# Autodesk Inventor assembly: GE-13027
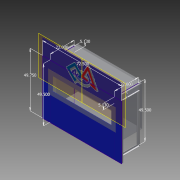
[picture p0: Inventor's stored thumbnail of the model, 180x180]
Saved by Autodesk Inventor 2013 (Build 170138000, 138)
## iProperties
Created: 2013-01-04
Part Number: GE-13027
Document SubType Name: Assembly
Designer: Phillip
Author: Phillip
## Documents named in this file (11)
- E:\Data Folder\FIRST 2013\FIRST KOP\FIRST Arena 2013\Feeder Goal Station\GE-13027.iam
- E:\Data Folder\FIRST 2013\FIRST KOP\FIRST Arena 2013\Feeder Goal Station\GE-13029.ipt
- E:\Data Folder\FIRST 2013\FIRST KOP\FIRST Arena 2013\Feeder Goal Station\GE-13013B.ipt
- E:\Data Folder\FIRST 2013\FIRST KOP\FIRST Arena 2013\Feeder Goal Station\GE-13013BLogo.ipt
- E:\Data Folder\FIRST 2013\FIRST KOP\FIRST Arena 2013\Feeder Goal Station\GE-13066.iam
- E:\Data Folder\FIRST 2013\FIRST KOP\FIRST Arena 2013\Feeder Goal Station\GE-13031.ipt
- E:\Data Folder\FIRST 2013\FIRST KOP\FIRST Arena 2013\Feeder Goal Station\box_middlegoal.ipt
- E:\Data Folder\FIRST 2013\FIRST KOP\FIRST Arena 2013\Feeder Goal Station\GE_13030.ipt
- E:\Data Folder\FIRST 2013\FIRST KOP\FIRST Arena 2013\Feeder Goal Station\GE-13065.iam
- E:\Data Folder\FIRST 2013\FIRST KOP\FIRST Arena 2013\Feeder Goal Station\GE-13064.ipt
- E:\Data Folder\FIRST 2013\FIRST KOP\FIRST Arena 2013\Feeder Goal Station\ReflectiveImage01.ipt
## Components (12 placed, 10 different names)
1. GE-13013B:1 — Flush:1, Mate:1, Flush:2, Flush:3, Flush:4
2. GE-13029:1 — Mate:17, Flush:7, Flush:9
3. GE-13013BLogo:1 — Flush:1, Mate:1, Flush:2, Mate:18, Flush:8, Flush:10, Flush:11, Mate:24, Angle:1
4. GE-13066:1 [sub-assembly] — Flush:5, Mate:10, Mate:14, Mate:15, Mate:16, Mate:21
5. GE-13066:2 [sub-assembly] — Mate:6, Mate:8, Flush:3, Flush:6, Mate:11, Mate:12, Mate:13, Mate:19, Mate:20
6. GE-13031:1 — Mate:5, Mate:8, Flush:6, Mate:22
7. box_middlegoal:1 — Mate:5, Mate:6, Flush:4, Flush:5, Mate:10
8. GE_13030:1 — Mate:11, Mate:12, Mate:13, Mate:17, Flush:7, Mate:23
9. GE_13030:2 — Mate:14, Mate:15, Mate:16
10. GE-13065:1 [sub-assembly] — Mate:18, Flush:8, Mate:19, Mate:20, Mate:21, Mate:22
11. GE-13064:1 — Mate:23, Flush:9
12. ReflectiveImage01:1 — Flush:10, Flush:11
## Relationships (31: Mate 19, Flush 11, Angle 1)
- Flush:1: GE-13013B:1 ↔ GE-13013BLogo:1
- Mate:1: GE-13013B:1 ↔ GE-13013BLogo:1
- Flush:2: GE-13013B:1 ↔ GE-13013BLogo:1
- Mate:5: GE-13031:1 ↔ box_middlegoal:1
- Mate:6: GE-13066:2 ↔ box_middlegoal:1
- Mate:8: GE-13066:2 ↔ GE-13031:1
- Flush:3: GE-13013B:1 ↔ GE-13066:2
- Flush:4 (-60.325 mm): GE-13013B:1 ↔ box_middlegoal:1
- Flush:5: GE-13066:1 ↔ box_middlegoal:1
- Mate:10: GE-13066:1 ↔ box_middlegoal:1
- Flush:6 (-9.525 mm): GE-13066:2 ↔ GE-13031:1
- Mate:11: GE-13066:2 ↔ GE_13030:1
- Mate:12: GE-13066:2 ↔ GE_13030:1
- Mate:13: GE-13066:2 ↔ GE_13030:1
- Mate:14: GE-13066:1 ↔ GE_13030:2
- Mate:15: GE-13066:1 ↔ GE_13030:2
- Mate:16: GE-13066:1 ↔ GE_13030:2
- Mate:17: GE-13029:1 ↔ GE_13030:1
- Flush:7 (46.0375 mm): GE-13029:1 ↔ GE_13030:1
- Mate:18: GE-13013BLogo:1 ↔ GE-13065:1
- Flush:8: GE-13013BLogo:1 ↔ GE-13065:1
- Mate:19: GE-13066:2 ↔ GE-13065:1
- Mate:20: GE-13066:2 ↔ GE-13065:1
- Mate:21: GE-13066:1 ↔ GE-13065:1
- Mate:22: GE-13031:1 ↔ GE-13065:1
- Mate:23: GE_13030:1 ↔ GE-13064:1
- Flush:9: GE-13029:1 ↔ GE-13064:1
- Flush:10: GE-13013BLogo:1 ↔ ReflectiveImage01:1
- Flush:11: GE-13013BLogo:1 ↔ ReflectiveImage01:1
- Mate:24: GE-13013BLogo:1
- Angle:1 (0 deg): GE-13013BLogo:1
